# Autodesk Inventor assembly: top gripper
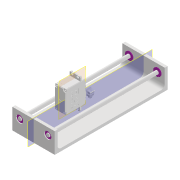
[picture p0: Inventor's stored thumbnail of the model, 180x180]
Saved by Autodesk Inventor 2020 (Build 240168000, 168)
## iProperties
Created: 2019-10-20
Part Number: top gripper
Document SubType Name: Assembly
Designer: ball
Author: ball
## Documents named in this file (6)
- C:\FTC\FTC8863CAD\2019 Robot\Collection\top gripper.iam
- C:\FTC\FTC8863CAD\RevRobotics\REV-41-1097.iam
- C:\FTC\FTC8863CAD\2019 Robot\Collection\Top grip collecter grip.ipt
- C:\FTC\FTC8863CAD\Actobotics\535 parts\535198.ipt
- C:\FTC\FTC8863CAD\Actobotics\634 parts\634088.ipt
- C:\FTC\FTC8863CAD\Actobotics\525 parts\525150 assembly.ipt
## Components (9 placed, 5 different names)
1. REV-41-1097:1 [sub-assembly] — Mate:1, Mate:2, Mate:3, Mate:14, Mate:15
2. Top grip collecter grip:1 — Mate:1, Mate:2, Mate:3, Mate:4, Mate:5, Mate:6, Mate:7, Mate:8, Mate:9, Mate:10, Mate:11, Flush:1, Flush:2, Mate:16, Mate:17, Mate:18
3. 535198:1 — Mate:4, Mate:5
4. 535198:2 — Mate:8, Mate:9, Mate:12
5. 535198:3 — Mate:6, Mate:7
6. 535198:4 — Mate:10, Mate:11, Mate:13
7. 634088:1 — Mate:13, Flush:2
8. 634088:2 — Mate:12, Flush:1
9. 525150 assembly:1 — Mate:14, Mate:15
## Relationships (20: Mate 18, Flush 2)
- Mate:1 (9.6266 mm): REV-41-1097:1 ↔ Top grip collecter grip:1
- Mate:2 (50.8 mm): REV-41-1097:1 ↔ Top grip collecter grip:1
- Mate:3 (8.4836 mm): REV-41-1097:1 ↔ Top grip collecter grip:1
- Mate:4: Top grip collecter grip:1 ↔ 535198:1
- Mate:5: Top grip collecter grip:1 ↔ 535198:1
- Mate:6: Top grip collecter grip:1 ↔ 535198:3
- Mate:7: Top grip collecter grip:1 ↔ 535198:3
- Mate:8: Top grip collecter grip:1 ↔ 535198:2
- Mate:9: Top grip collecter grip:1 ↔ 535198:2
- Mate:10: Top grip collecter grip:1 ↔ 535198:4
- Mate:11: Top grip collecter grip:1 ↔ 535198:4
- Mate:12: 535198:2 ↔ 634088:2
- Mate:13: 535198:4 ↔ 634088:1
- Flush:1: Top grip collecter grip:1 ↔ 634088:2
- Flush:2: Top grip collecter grip:1 ↔ 634088:1
- Mate:14: REV-41-1097:1 ↔ 525150 assembly:1
- Mate:15: REV-41-1097:1 ↔ 525150 assembly:1
- Mate:16: Top grip collecter grip:1
- Mate:17: Top grip collecter grip:1
- Mate:18: Top grip collecter grip:1
